# Autodesk Inventor assembly: Gear assembly
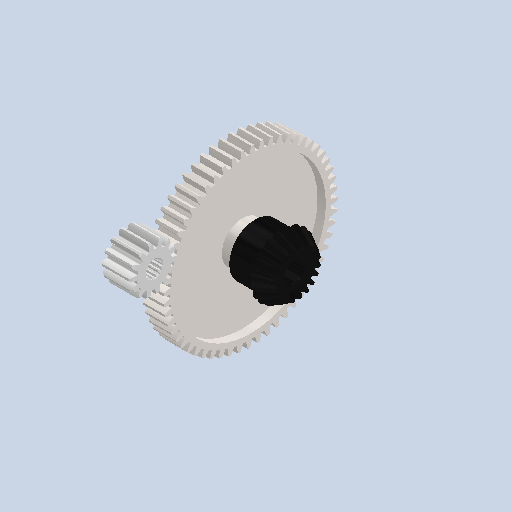
[picture p0: Inventor's stored thumbnail of the model, 512x512]
Saved by Autodesk Inventor 2023 (Build 270158030, 158C)
## iProperties
Created: 2022-10-20
Part Number: Gear assembly
Document SubType Name: Assembly
Designer: cjj5381
Author: cjj5381
## Documents named in this file (4)
- V:\Robtotics\Gears\Gear assembly.iam
- V:\Robtotics\Gears\am-2621_20t_1-25mod_bevel_gear.ipt
- V:\Robtotics\Gears\am-3822 56T 20DP 500hex 375 FW.ipt
- V:\Robtotics\Gears\am-4147 14T 20DP Gear Spline Bore Falcon 500 Pinion.ipt
## Components (3 placed, 3 different names)
1. am-2621_20t_1-25mod_bevel_gear:1 — Mate:3, Mate:7
2. am-3822 56T 20DP 500hex 375 FW:1 — Mate:3, Tangent:2, Rotation:1, Mate:6, Mate:7
3. am-4147 14T 20DP Gear Spline Bore Falcon 500 Pinion:1 — Tangent:2, Rotation:1, Mate:4, Mate:5
## Relationships (7: Mate 5, Tangent 1, RelateRotation 1)
- Mate:3: am-2621_20t_1-25mod_bevel_gear:1 ↔ am-3822 56T 20DP 500hex 375 FW:1
- Tangent:2: am-3822 56T 20DP 500hex 375 FW:1 ↔ am-4147 14T 20DP Gear Spline Bore Falcon 500 Pinion:1
- Rotation:1 [RelateRotation] (1 ul): am-3822 56T 20DP 500hex 375 FW:1 ↔ am-4147 14T 20DP Gear Spline Bore Falcon 500 Pinion:1
- Mate:4: am-4147 14T 20DP Gear Spline Bore Falcon 500 Pinion:1
- Mate:5: am-4147 14T 20DP Gear Spline Bore Falcon 500 Pinion:1
- Mate:6: am-3822 56T 20DP 500hex 375 FW:1
- Mate:7: am-2621_20t_1-25mod_bevel_gear:1 ↔ am-3822 56T 20DP 500hex 375 FW:1
